# Autodesk Inventor assembly: Universal Joint
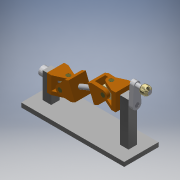
[picture p0: Inventor's stored thumbnail of the model, 180x180]
Saved by Autodesk Inventor 2017 (Build 210142000, 142)
## iProperties
Created: 2014-03-04
Part Number: Universal Joint
Document SubType Name: Assembly
Designer: John
Author: John
## Documents named in this file (9)
- C:\Users\John Helfen\Desktop\Ex_Files_Invent_2016_EssT\Ex_Files_Invent_2016_EssT\Exercise Files\14_Using constraints to position parts\14_01\Universal Joint.iam
- C:\Users\John Helfen\Desktop\Ex_Files_Invent_2016_EssT\Ex_Files_Invent_2016_EssT\Exercise Files\14_Using constraints to position parts\14_01\base.ipt
- C:\Users\John Helfen\Desktop\Ex_Files_Invent_2016_EssT\Ex_Files_Invent_2016_EssT\Exercise Files\14_Using constraints to position parts\14_01\Connector.ipt
- C:\Users\John Helfen\Desktop\Ex_Files_Invent_2016_EssT\Ex_Files_Invent_2016_EssT\Exercise Files\14_Using constraints to position parts\14_01\Joint.ipt
- C:\Users\John Helfen\Desktop\Ex_Files_Invent_2016_EssT\Ex_Files_Invent_2016_EssT\Exercise Files\14_Using constraints to position parts\14_01\Crank Rod.ipt
- C:\Users\John Helfen\Desktop\Ex_Files_Invent_2016_EssT\Ex_Files_Invent_2016_EssT\Exercise Files\14_Using constraints to position parts\14_01\Crank Handle.ipt
- C:\Users\John Helfen\Desktop\Ex_Files_Invent_2016_EssT\Ex_Files_Invent_2016_EssT\Exercise Files\14_Using constraints to position parts\14_01\Pin.ipt
- C:\Users\John Helfen\Desktop\Ex_Files_Invent_2016_EssT\Ex_Files_Invent_2016_EssT\Exercise Files\14_Using constraints to position parts\14_01\Universal Shaft.iam
- C:\Users\John Helfen\Desktop\Ex_Files_Invent_2016_EssT\Ex_Files_Invent_2016_EssT\Exercise Files\14_Using constraints to position parts\14_01\Handle.ipt
## Components (19 placed, 9 different names)
1. base:1 — Mate:1, Mate:2, Mate:9, Mate:10, Mate:15, Mate:16, Angle:3 - DRIVE THIS
2. Connector:1 — Mate:3, Mate:4
3. Connector:2 — Mate:5, Mate:6
4. Joint:1 — Mate:1, Mate:2, Mate:3, Mate:4, Flush:3, Angle:1, Insert:1, Insert:2
5. Joint:2 — Mate:5, Mate:6, Mate:9, Mate:10, Flush:4, Angle:2, Insert:5, Insert:8
6. Crank Rod:1 — Mate:15, Flush:3, Flush:5, Mate:17
7. Crank Rod:2 — Flush:4, Mate:16, Flush:6, Mate:18
8. Crank Handle:1 - DRIVE — Flush:5, Mate:17, Angle:1, Angle:3 - DRIVE THIS, Mate:21, Mate:22
9. Crank Handle:2 — Flush:6, Angle:2, Mate:18
10. Pin:1 — Insert:1
11. Pin:2 — Mate:19, Flush:7
12. Pin:3
13. Pin:4 — Insert:2
14. Pin:5
15. Pin:6 — Insert:8
16. Pin:7 — Flush:8, Mate:20
17. Pin:8 — Insert:5
18. Universal Shaft:1 [sub-assembly] — Mate:19, Flush:7, Flush:8, Mate:20
19. Handle:1 — Mate:21, Mate:22
## Relationships (29: Mate 16, Flush 6, Insert 4, Angle 3)
- Mate:1: base:1 ↔ Joint:1
- Mate:2: base:1 ↔ Joint:1
- Mate:3: Connector:1 ↔ Joint:1
- Mate:4 (1.27 mm): Connector:1 ↔ Joint:1
- Mate:5: Connector:2 ↔ Joint:2
- Mate:6 (1.27 mm): Connector:2 ↔ Joint:2
- Mate:9: base:1 ↔ Joint:2
- Mate:10: base:1 ↔ Joint:2
- Mate:15: base:1 ↔ Crank Rod:1
- Flush:3: Joint:1 ↔ Crank Rod:1
- Flush:4: Joint:2 ↔ Crank Rod:2
- Mate:16: base:1 ↔ Crank Rod:2
- Flush:5: Crank Rod:1 ↔ Crank Handle:1 - DRIVE
- Mate:17: Crank Rod:1 ↔ Crank Handle:1 - DRIVE
- Angle:1 (0 deg): Joint:1 ↔ Crank Handle:1 - DRIVE
- Flush:6: Crank Rod:2 ↔ Crank Handle:2
- Angle:2 (45 deg): Joint:2 ↔ Crank Handle:2
- Mate:18: Crank Rod:2 ↔ Crank Handle:2
- Insert:1: Joint:1 ↔ Pin:1
- Insert:2: Joint:1 ↔ Pin:4
- Insert:5: Joint:2 ↔ Pin:8
- Insert:8: Joint:2 ↔ Pin:6
- Angle:3 - DRIVE THIS (180 deg): base:1 ↔ Crank Handle:1 - DRIVE
- Mate:19: Pin:2 ↔ Universal Shaft:1
- Flush:7: Pin:2 ↔ Universal Shaft:1
- Flush:8: Pin:7 ↔ Universal Shaft:1
- Mate:20: Pin:7 ↔ Universal Shaft:1
- Mate:21: Crank Handle:1 - DRIVE ↔ Handle:1
- Mate:22: Crank Handle:1 - DRIVE ↔ Handle:1
